# Autodesk Inventor assembly: Konarm_3_przegub_v2
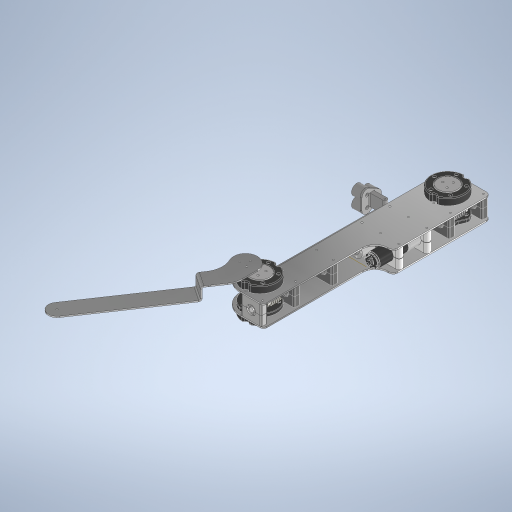
[picture p0: Inventor's stored thumbnail of the model, 512x512]
Saved by Autodesk Inventor 2023 (Build 270158000, 158)
## iProperties
Created: 2023-01-27
Part Number: Konarm_3_przegub_v2
Document SubType Name: Assembly
Designer: Kamil
Mass: 929.155 g
Surface Area: 4430.92 cm^2
Volume: 901.223 cm^3
Density: 1.03099 g/cm^3
Author: Kamil
## Documents named in this file (20)
- C:\Users\Kamil\Desktop\KONARM\konarm 3 przegub\Konarm_3_przegub_v2.iam
- C:\Users\Kamil\Desktop\KONARM\konarm 3 przegub\blacha.ipt
- C:\Users\Kamil\Desktop\KONARM\konarm 3 przegub\koszyczek.ipt
- C:\Users\Kamil\Desktop\KONARM\konarm 3 przegub\kolnierz wewnetrzny.ipt
- C:\Users\Kamil\Desktop\KONARM\konarm 3 przegub\Złożenie2.STEP.ipt
- C:\Users\Kamil\Desktop\KONARM\konarm 3 przegub\Faulhaber 3272G012C R.ipt
- C:\Users\Kamil\Desktop\KONARM\konarm 3 przegub\os_napedowa.ipt
- C:\Users\Kamil\Desktop\KONARM\konarm 3 przegub\Os.ipt
- C:\Users\Kamil\Desktop\KONARM\konarm 3 przegub\Os_lewa.ipt
- C:\Users\Kamil\Desktop\KONARM\konarm 3 przegub\kółko.ipt
- C:\Users\Kamil\Desktop\KONARM\konarm 3 przegub\ball bearing(6006).ipt
- C:\Users\Kamil\Desktop\KONARM\konarm 3 przegub\FAG BALL BEARING 6200.ipt
- C:\Users\Kamil\Desktop\KONARM\konarm 3 przegub\Uchwyt_na_lozysko_poli.ipt
- C:\Users\Kamil\Desktop\KONARM\konarm 3 przegub\blacha_MIR.ipt
- C:\Users\Kamil\Desktop\KONARM\konarm 3 przegub\blacha_2.ipt
- C:\Users\Kamil\Desktop\KONARM\konarm 3 przegub\blacha_2_MIR.ipt
- C:\Users\Kamil\Desktop\KONARM\konarm 3 przegub\Ariadna-Electromagnet_mount_v2.ipt
- C:\Users\Kamil\Desktop\KONARM\konarm 3 przegub\wspornik.ipt
- C:\Users\Kamil\Desktop\KONARM\konarm 3 przegub\Złożenie2.STEP_MIR.ipt
- C:\Users\Kamil\Desktop\KONARM\konarm 3 przegub\Uchwyt_silnika_podwojny.ipt
## Components (50 placed, 19 different names)
1. blacha:2 — Mate:4, Mate:6, Mate:7, Mate:8, Mate:9, Mate:16, Mate:17, Mate:18, Mate:22, Mate:50, Mate:52, Flush:2, Mate:55, Mate:96, Mate:98, Mate:100, Mate:104, Mate:105, Mate:109, Mate:110, Mate:112, Mate:113, Mate:114, Mate:118, Mate:119, Mate:126, Mate:134, Flush:11, Flush:12
2. koszyczek:1 — Mate:84, Mate:85, Mate:86
3. koszyczek:2 — Mate:7, Mate:8, Mate:9
4. kolnierz wewnetrzny:1 — Mate:16, Mate:17, Mate:18, Mate:54
5. kolnierz wewnetrzny:2 — Mate:80, Mate:81, Mate:82, Mate:83
6. Złożenie2.STEP:1 — Mate:27, Mate:28, Zestawiające:145
7. Faulhaber 3272G012C R:1 — Mate:32, Mate:33, Flush:9
8. os_napedowa:1 — Mate:27, Mate:29, Mate:30, Mate:31, Mate:32, Mate:33, Mate:51, Mate:53, Mate:56, Mate:63, Mate:64, Mate:65, Flush:6
9. Os:1 — Mate:19, Mate:20, Mate:23, Mate:76, Mate:81, Zestawiające:149, Zestawiające:154, Zestawiające:155
10. Os_lewa:1 — Mate:21, Mate:22, Mate:23, Mate:28, Mate:76, Zestawiające:149, Zestawiające:150, Zestawiające:151
11. ball bearing(6006):1 — Mate:4, Mate:6, Mate:21, Zestawiające:145, Zestawiające:148
12. ball bearing(6006):2 — Mate:19, Mate:20, Mate:77, Mate:85, Zestawiające:152, Zestawiające:153
13. FAG BALL BEARING 6200:1 — Mate:31, Mate:57
14. FAG BALL BEARING 6200:2 — Mate:29, Mate:58
15. FAG BALL BEARING 6200:3 — Mate:30, Mate:59
16. Uchwyt_na_lozysko_poli:1 — Mate:50, Mate:51, Flush:2, Mate:59, Flush:3
17. Uchwyt_na_lozysko_poli:2 — Mate:55, Mate:56, Mate:57, Flush:5
18. Uchwyt_na_lozysko_poli:3 — Mate:65, Flush:5, Mate:71
19. Uchwyt_na_lozysko_poli:4 — Mate:64, Flush:4, Mate:79
20. Uchwyt_na_lozysko_poli:5 — Mate:63, Flush:3, Mate:74, Flush:6
21. Uchwyt_na_lozysko_poli:6 — Mate:52, Mate:53, Mate:54, Mate:58, Flush:4
22. blacha_MIR:1 — Mate:71, Mate:74, Mate:77, Mate:79, Mate:80, Mate:82, Mate:83, Mate:84, Mate:86, Mate:95, Mate:97, Mate:103, Mate:106, Flush:10, Mate:115, Mate:116, Mate:117, Mate:120, Mate:121, Mate:128, Mate:135, Mate:138, Flush:11, Flush:12
23. blacha_2:1 — Mate:91, Mate:92, Mate:93, Zestawiające:156, Zestawiające:159
24. blacha_2_MIR:1 — Mate:91, Flush:7, Zestawiające:157, Zestawiające:158
25. Ariadna-Electromagnet_mount_v2:1 — Mate:92, Mate:93
26. wspornik:1 — Flush:7
27. Złożenie2.STEP_MIR:2 — Mate:99, Mate:100, Mate:102
28. Faulhaber 3272G012C R:2 — Mate:102, Mate:107, Mate:108, Flush:9, Mate:111
29. Uchwyt_na_lozysko_poli:7 — Mate:95, Mate:97, Mate:99, Mate:107, Mate:130
30. Uchwyt_na_lozysko_poli:8 — Mate:96, Mate:98, Mate:131
31. Uchwyt_na_lozysko_poli:9 — Mate:103, Mate:106, Mate:108, Mate:132, Mate:133
32. Uchwyt_na_lozysko_poli:10 — Mate:104, Mate:105
33. Uchwyt_silnika_podwojny:1 — Flush:10
34. Uchwyt_silnika_podwojny:2 — Mate:112, Mate:113, Mate:114
35. Uchwyt_silnika_podwojny:3 — Mate:109, Mate:110, Mate:111
36. Uchwyt_silnika_podwojny:4 — Mate:115, Mate:116, Mate:117
37. koszyczek:3 — Mate:126, Mate:127, Mate:139
38. ball bearing(6006):3 — Mate:120, Mate:121, Mate:124, Mate:125, Mate:129, Mate:142, Zestawiające:146
39. kółko:3 — Mate:141, Mate:142, Mate:144, Zestawiające:146, Zestawiające:161, Zestawiające:162
40. Os_lewa:2 — Mate:122, Mate:123, Mate:136, Mate:140, Zestawiające:160, Zestawiające:163, Zestawiające:164
41. Os:2 — Mate:124, Mate:125, Mate:137, Mate:141, Zestawiające:160, Zestawiające:161, Zestawiające:162
42. kolnierz wewnetrzny:3 — Mate:134, Mate:136, Mate:139
43. koszyczek:4 — Mate:128, Mate:129, Mate:138
44. kolnierz wewnetrzny:4 — Mate:135, Mate:137
45. ball bearing(6006):4 — Mate:118, Mate:119, Mate:122, Mate:123, Mate:127, Mate:143, Zestawiające:147
46. kółko:4 — Mate:140, Mate:143, Mate:144, Zestawiające:147, Zestawiające:163, Zestawiające:164
47. FAG BALL BEARING 6200:4 — Mate:130, Mate:131
48. FAG BALL BEARING 6200:5 — Mate:132, Mate:133
49. kółko:5 — Zestawiające:148, Zestawiające:150, Zestawiające:151, Zestawiające:156, Zestawiające:159
50. kółko:6 — Zestawiające:152, Zestawiające:153, Zestawiające:154, Zestawiające:155, Zestawiające:157, Zestawiające:158
## Relationships (127: Mate 117, Flush 10)
- Mate:4: blacha:2 ↔ ball bearing(6006):1
- Mate:6: blacha:2 ↔ ball bearing(6006):1
- Mate:7: blacha:2 ↔ koszyczek:2
- Mate:8: blacha:2 ↔ koszyczek:2
- Mate:9: blacha:2 ↔ koszyczek:2
- Mate:16: blacha:2 ↔ kolnierz wewnetrzny:1
- Mate:17: blacha:2 ↔ kolnierz wewnetrzny:1
- Mate:18: blacha:2 ↔ kolnierz wewnetrzny:1
- Mate:19: Os:1 ↔ ball bearing(6006):2
- Mate:20: Os:1 ↔ ball bearing(6006):2
- Mate:21: Os_lewa:1 ↔ ball bearing(6006):1
- Mate:22: blacha:2 ↔ Os_lewa:1
- Mate:23: Os:1 ↔ Os_lewa:1
- Mate:27: Złożenie2.STEP:1 ↔ os_napedowa:1
- Mate:28: Złożenie2.STEP:1 ↔ Os_lewa:1
- Mate:29: os_napedowa:1 ↔ FAG BALL BEARING 6200:2
- Mate:30: os_napedowa:1 ↔ FAG BALL BEARING 6200:3
- Mate:31: os_napedowa:1 ↔ FAG BALL BEARING 6200:1
- Mate:32: Faulhaber 3272G012C R:1 ↔ os_napedowa:1
- Mate:33 (5 mm): Faulhaber 3272G012C R:1 ↔ os_napedowa:1
- Mate:50: blacha:2 ↔ Uchwyt_na_lozysko_poli:1
- Mate:51: os_napedowa:1 ↔ Uchwyt_na_lozysko_poli:1
- Mate:52: blacha:2 ↔ Uchwyt_na_lozysko_poli:6
- Mate:53: os_napedowa:1 ↔ Uchwyt_na_lozysko_poli:6
- Flush:2: blacha:2 ↔ Uchwyt_na_lozysko_poli:1
- Mate:54 (1.14 mm): kolnierz wewnetrzny:1 ↔ Uchwyt_na_lozysko_poli:6
- Mate:55: blacha:2 ↔ Uchwyt_na_lozysko_poli:2
- Mate:56: os_napedowa:1 ↔ Uchwyt_na_lozysko_poli:2
- Mate:57: FAG BALL BEARING 6200:1 ↔ Uchwyt_na_lozysko_poli:2
- Mate:58: FAG BALL BEARING 6200:2 ↔ Uchwyt_na_lozysko_poli:6
- Mate:59: FAG BALL BEARING 6200:3 ↔ Uchwyt_na_lozysko_poli:1
- Mate:63: os_napedowa:1 ↔ Uchwyt_na_lozysko_poli:5
- Mate:64: os_napedowa:1 ↔ Uchwyt_na_lozysko_poli:4
- Mate:65: os_napedowa:1 ↔ Uchwyt_na_lozysko_poli:3
- Flush:3: Uchwyt_na_lozysko_poli:1 ↔ Uchwyt_na_lozysko_poli:5
- Flush:4: Uchwyt_na_lozysko_poli:4 ↔ Uchwyt_na_lozysko_poli:6
- Flush:5: Uchwyt_na_lozysko_poli:2 ↔ Uchwyt_na_lozysko_poli:3
- Mate:71: Uchwyt_na_lozysko_poli:3 ↔ blacha_MIR:1
- Mate:74: Uchwyt_na_lozysko_poli:5 ↔ blacha_MIR:1
- Mate:76: Os:1 ↔ Os_lewa:1
- Mate:77: ball bearing(6006):2 ↔ blacha_MIR:1
- Mate:79: Uchwyt_na_lozysko_poli:4 ↔ blacha_MIR:1
- Mate:80: kolnierz wewnetrzny:2 ↔ blacha_MIR:1
- Mate:81: kolnierz wewnetrzny:2 ↔ Os:1
- Mate:82: kolnierz wewnetrzny:2 ↔ blacha_MIR:1
- Mate:83: kolnierz wewnetrzny:2 ↔ blacha_MIR:1
- Mate:84: koszyczek:1 ↔ blacha_MIR:1
- Mate:85: koszyczek:1 ↔ ball bearing(6006):2
- Mate:86: koszyczek:1 ↔ blacha_MIR:1
- Mate:91: blacha_2:1 ↔ blacha_2_MIR:1
- Mate:92: blacha_2:1 ↔ Ariadna-Electromagnet_mount_v2:1
- Flush:6: os_napedowa:1 ↔ Uchwyt_na_lozysko_poli:5
- Mate:93 (2.5 mm): blacha_2:1 ↔ Ariadna-Electromagnet_mount_v2:1
- Flush:7: blacha_2_MIR:1 ↔ wspornik:1
- Mate:95: blacha_MIR:1 ↔ Uchwyt_na_lozysko_poli:7
- Mate:96: blacha:2 ↔ Uchwyt_na_lozysko_poli:8
- Mate:97: blacha_MIR:1 ↔ Uchwyt_na_lozysko_poli:7
- Mate:98: blacha:2 ↔ Uchwyt_na_lozysko_poli:8
- Mate:99: Złożenie2.STEP_MIR:2 ↔ Uchwyt_na_lozysko_poli:7
- Mate:100: blacha:2 ↔ Złożenie2.STEP_MIR:2
- Mate:102: Złożenie2.STEP_MIR:2 ↔ Faulhaber 3272G012C R:2
- Mate:103: blacha_MIR:1 ↔ Uchwyt_na_lozysko_poli:9
- Mate:104: blacha:2 ↔ Uchwyt_na_lozysko_poli:10
- Mate:105: blacha:2 ↔ Uchwyt_na_lozysko_poli:10
- Mate:106: blacha_MIR:1 ↔ Uchwyt_na_lozysko_poli:9
- Mate:107: Faulhaber 3272G012C R:2 ↔ Uchwyt_na_lozysko_poli:7
- Mate:108: Faulhaber 3272G012C R:2 ↔ Uchwyt_na_lozysko_poli:9
- Flush:9: Faulhaber 3272G012C R:1 ↔ Faulhaber 3272G012C R:2
- Flush:10: blacha_MIR:1 ↔ Uchwyt_silnika_podwojny:1
- Mate:109: blacha:2 ↔ Uchwyt_silnika_podwojny:3
- Mate:110: blacha:2 ↔ Uchwyt_silnika_podwojny:3
- Mate:111: Faulhaber 3272G012C R:2 ↔ Uchwyt_silnika_podwojny:3
- Mate:112: blacha:2 ↔ Uchwyt_silnika_podwojny:2
- Mate:113: blacha:2 ↔ Uchwyt_silnika_podwojny:2
- Mate:114: blacha:2 ↔ Uchwyt_silnika_podwojny:2
- Mate:115: blacha_MIR:1 ↔ Uchwyt_silnika_podwojny:4
- Mate:116: blacha_MIR:1 ↔ Uchwyt_silnika_podwojny:4
- Mate:117: blacha_MIR:1 ↔ Uchwyt_silnika_podwojny:4
- Mate:118: blacha:2 ↔ ball bearing(6006):4
- Mate:119: blacha:2 ↔ ball bearing(6006):4
- Mate:120: blacha_MIR:1 ↔ ball bearing(6006):3
- Mate:121: blacha_MIR:1 ↔ ball bearing(6006):3
- Mate:122: Os_lewa:2 ↔ ball bearing(6006):4
- Mate:123: Os_lewa:2 ↔ ball bearing(6006):4
- Mate:124: ball bearing(6006):3 ↔ Os:2
- Mate:125: ball bearing(6006):3 ↔ Os:2
- Mate:126: blacha:2 ↔ koszyczek:3
- Mate:127: koszyczek:3 ↔ ball bearing(6006):4
- Mate:128: blacha_MIR:1 ↔ koszyczek:4
- Mate:129: ball bearing(6006):3 ↔ koszyczek:4
- Mate:130: Uchwyt_na_lozysko_poli:7 ↔ FAG BALL BEARING 6200:4
- Mate:131: Uchwyt_na_lozysko_poli:8 ↔ FAG BALL BEARING 6200:4
- Mate:132: Uchwyt_na_lozysko_poli:9 ↔ FAG BALL BEARING 6200:5
- Mate:133: Uchwyt_na_lozysko_poli:9 ↔ FAG BALL BEARING 6200:5
- Mate:134: blacha:2 ↔ kolnierz wewnetrzny:3
- Mate:135: blacha_MIR:1 ↔ kolnierz wewnetrzny:4
- Mate:136: Os_lewa:2 ↔ kolnierz wewnetrzny:3
- Mate:137: Os:2 ↔ kolnierz wewnetrzny:4
- Mate:138: blacha_MIR:1 ↔ koszyczek:4
- Mate:139: koszyczek:3 ↔ kolnierz wewnetrzny:3
- Mate:140: Os_lewa:2 ↔ kółko:4
- Mate:141: kółko:3 ↔ Os:2
- Mate:142: ball bearing(6006):3 ↔ kółko:3
- Mate:143: ball bearing(6006):4 ↔ kółko:4
- Mate:144: kółko:3 ↔ kółko:4
- Flush:11: blacha:2 ↔ blacha_MIR:1
- Flush:12: blacha:2 ↔ blacha_MIR:1
- Zestawiające:145 [Mate]: Złożenie2.STEP:1 ↔ ball bearing(6006):1
- Zestawiające:146 [Mate]: ball bearing(6006):3 ↔ kółko:3
- Zestawiające:147 [Mate]: ball bearing(6006):4 ↔ kółko:4
- Zestawiające:148 [Mate]: ball bearing(6006):1 ↔ kółko:5
- Zestawiające:149 [Mate]: Os:1 ↔ Os_lewa:1
- Zestawiające:150 [Mate]: Os_lewa:1 ↔ kółko:5
- Zestawiające:151 [Mate]: Os_lewa:1 ↔ kółko:5
- Zestawiające:152 [Mate]: ball bearing(6006):2 ↔ kółko:6
- Zestawiające:153 [Mate]: ball bearing(6006):2 ↔ kółko:6
- Zestawiające:154 [Mate]: Os:1 ↔ kółko:6
- Zestawiające:155 [Mate]: Os:1 ↔ kółko:6
- Zestawiające:156 [Mate]: blacha_2:1 ↔ kółko:5
- Zestawiające:157 [Mate]: blacha_2_MIR:1 ↔ kółko:6
- Zestawiające:158 [Mate]: blacha_2_MIR:1 ↔ kółko:6
- Zestawiające:159 [Mate]: blacha_2:1 ↔ kółko:5
- Zestawiające:160 [Mate]: Os_lewa:2 ↔ Os:2
- Zestawiające:161 [Mate]: kółko:3 ↔ Os:2
- Zestawiające:162 [Mate]: kółko:3 ↔ Os:2
- Zestawiające:163 [Mate]: Os_lewa:2 ↔ kółko:4
- Zestawiające:164 [Mate]: Os_lewa:2 ↔ kółko:4
